# Autodesk Inventor assembly: Assembly cajon grande
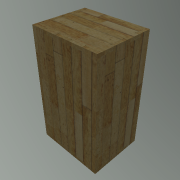
[picture p0: Inventor's stored thumbnail of the model, 180x180]
Saved by Autodesk Inventor 2015 (Build 190159000, 159)
## iProperties
Created: 2016-01-28
Part Number: Assembly cajon grande
Document SubType Name: Assembly
Designer: 172406
Author: 172406
## Documents named in this file (4)
- H:\3d\Assembly cajon grande.iam
- H:\3d\cajon abajo.ipt
- H:\3d\cajon front grande.ipt
- H:\3d\cajon lat grande.ipt
## Components (5 placed, 3 different names)
1. cajon front grande:1 — Flush:3, Mate:3, Flush:4
2. cajon lat grande:1 — Mate:4, Flush:5
3. cajon abajo:2 — Flush:1, Flush:2, Mate:1, Mate:2, Flush:3, Mate:3, Flush:4, Flush:6, Flush:7, Mate:5
4. cajon front grande:2 — Flush:1, Flush:2, Mate:1, Mate:2, Mate:4, Flush:5
5. cajon lat grande:2 — Flush:6, Flush:7, Mate:5
## Relationships (12: Flush 7, Mate 5)
- Flush:1: cajon abajo:2 ↔ cajon front grande:2
- Flush:2: cajon abajo:2 ↔ cajon front grande:2
- Mate:1: cajon abajo:2 ↔ cajon front grande:2
- Mate:2: cajon abajo:2 ↔ cajon front grande:2
- Flush:3: cajon front grande:1 ↔ cajon abajo:2
- Mate:3: cajon front grande:1 ↔ cajon abajo:2
- Flush:4: cajon front grande:1 ↔ cajon abajo:2
- Mate:4: cajon lat grande:1 ↔ cajon front grande:2
- Flush:5: cajon lat grande:1 ↔ cajon front grande:2
- Flush:6: cajon abajo:2 ↔ cajon lat grande:2
- Flush:7: cajon abajo:2 ↔ cajon lat grande:2
- Mate:5: cajon abajo:2 ↔ cajon lat grande:2
